# Autodesk Inventor assembly: Zlozenie_268533
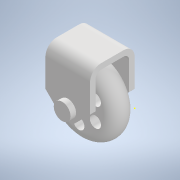
[picture p0: Inventor's stored thumbnail of the model, 180x180]
Saved by Autodesk Inventor 2022 (Build 260153000, 153)
## iProperties
Created: 2024-01-21
Part Number: Zlozenie_268533
Document SubType Name: Assembly
Designer: mateu
Author: mateu
## Documents named in this file (5)
- C:\Users\mateu\OneDrive\Dokumenty\Inventor\268533_podejscie2\Zlozenie_268533.iam
- C:\Users\mateu\OneDrive\Dokumenty\Inventor\268533_podejscie2\Blacha.ipt
- C:\Users\mateu\OneDrive\Dokumenty\Inventor\268533_podejscie2\Kolo.ipt
- C:\Users\mateu\OneDrive\Dokumenty\Inventor\268533_podejscie2\Trzemień.ipt
- C:\Users\mateu\OneDrive\Dokumenty\Inventor\Content Center Files\R2022\en-US\ISO 7434(2)\ISO 7434 - M3 x 8ISO.ipt
## Components (4 placed, 4 different names)
1. Blacha:1 — Mate:1, Mate:2, Insert:3
2. Kolo:1 — Mate:1, Insert:1, Mate:2, Insert:2
3. Trzemień:1 — Insert:1, Insert:2, Insert:3, Mate:3
4. ISO 7434 M3x8:2 — Mate:3
## Relationships (6: Mate 3, Insert 3)
- Mate:1: Blacha:1 ↔ Kolo:1
- Insert:1: Kolo:1 ↔ Trzemień:1
- Mate:2: Blacha:1 ↔ Kolo:1
- Insert:2 (50.8 mm): Kolo:1 ↔ Trzemień:1
- Insert:3: Blacha:1 ↔ Trzemień:1
- Mate:3: Trzemień:1 ↔ ISO 7434 M3x8:2
